# Autodesk Inventor assembly: Turret Columb Assembly
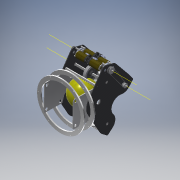
[picture p0: Inventor's stored thumbnail of the model, 180x180]
Saved by Autodesk Inventor 2019.4 (Build 234330000, 330)
## iProperties
Created: 2020-01-18
Part Number: Turret Columb Assembly
Document SubType Name: Assembly
Designer: admin
Mass: 1.34727e+06 g
Surface Area: 13984.7 cm^2
Volume: 9073.08 cm^3
Density: 148.491 g/cm^3
Author: admin
## Documents named in this file (4)
- C:\Users\admin\Desktop\FRC 2020 Engineering\GitHub\7738-2020\Robot V2\Turret Columb Assembly\Turret Columb Assembly.iam
- C:\Users\admin\Desktop\FRC 2020 Engineering\GitHub\7738-2020\Robot V2\Turret\Turret Assembly.iam
- C:\Users\admin\Desktop\FRC 2020 Engineering\GitHub\7738-2020\Robot V2\Turret Columb Assembly\Column Plate.ipt
- C:\Users\admin\Desktop\FRC 2020 Engineering\GitHub\7738-2020\Robot V2\Turret Columb Assembly\Slewing Bearing.ipt
## Components (5 placed, 3 different names)
1. Turret Assembly:1 [sub-assembly] — Angle:1, Mate:1, Mate:4, Mate:5, Mate:6
2. Column Plate:1 — Mate:2, Mate:3, Mate:5
3. Column Plate:2 — Mate:2, Mate:3, Mate:4, Mate:6
4. Slewing Bearing:1 — Mate:8
5. Slewing Bearing:2 — Mate:7, Mate:8
## Relationships (9: Mate 8, Angle 1)
- Angle:1 (60 deg): Turret Assembly:1
- Mate:1: Turret Assembly:1
- Mate:2: Column Plate:1 ↔ Column Plate:2
- Mate:3: Column Plate:1 ↔ Column Plate:2
- Mate:4 (5 mm): Turret Assembly:1 ↔ Column Plate:2
- Mate:5 (5 mm): Turret Assembly:1 ↔ Column Plate:1
- Mate:6: Turret Assembly:1 ↔ Column Plate:2
- Mate:7: Slewing Bearing:2
- Mate:8: Slewing Bearing:1 ↔ Slewing Bearing:2
